# Autodesk Inventor assembly: realsenses_plate_v2.ipt
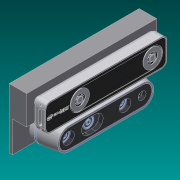
[picture p0: Inventor's stored thumbnail of the model, 180x180]
Saved by Autodesk Inventor 2020 (Build 240168000, 168)
## iProperties
Created: 2021-06-14
Part Number: realsenses_plate_v2.ipt
Document SubType Name: Assembly
Designer: Петров Иван
Mass: 324.425 g
Surface Area: 528.467 cm^2
Volume: 128.237 cm^3
Density: 2.52989 g/cm^3
Author: Петров Иван
## Documents named in this file (4)
- E:\IVAN\Ivan_desktop\Kvantorium\Projects\RoboPatrol\design\tests\realsenses_plate_v2.ipt.iam
- E:\IVAN\Ivan_desktop\Kvantorium\Projects\RoboPatrol\design\standart_components\Realsense\D200\Intel RealSense T265.iam
- E:\IVAN\Ivan_desktop\Kvantorium\Projects\RoboPatrol\design\standart_components\Realsense\D400\IntelRealsense_D435_Multibody.ipt
- E:\IVAN\Ivan_desktop\Kvantorium\Projects\RoboPatrol\design\tests\realsenses_plate_2.ipt
## Components (3 placed, 3 different names)
1. Intel RealSense T265:1 [sub-assembly] — Заподлицо:1, Совмещение:1, Совмещение:2
2. IntelRealsense_D435_Multibody:1 — Заподлицо:1, Совмещение:1, Совмещение:2, Совмещение:3, Совмещение:4, Совмещение:5
3. realsenses_plate_2:2 — Совмещение:3, Совмещение:4, Совмещение:5
## Relationships (6: Mate 5, Flush 1)
- Заподлицо:1 [Flush]: Intel RealSense T265:1 ↔ IntelRealsense_D435_Multibody:1
- Совмещение:1 [Mate]: Intel RealSense T265:1 ↔ IntelRealsense_D435_Multibody:1
- Совмещение:2 [Mate]: Intel RealSense T265:1 ↔ IntelRealsense_D435_Multibody:1
- Совмещение:3 [Mate]: IntelRealsense_D435_Multibody:1 ↔ realsenses_plate_2:2
- Совмещение:4 [Mate]: IntelRealsense_D435_Multibody:1 ↔ realsenses_plate_2:2
- Совмещение:5 [Mate]: IntelRealsense_D435_Multibody:1 ↔ realsenses_plate_2:2
